# Autodesk Inventor assembly: Maintenance_stand
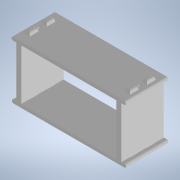
[picture p0: Inventor's stored thumbnail of the model, 180x180]
Saved by Autodesk Inventor 2020.2 (Build 242310000, 310)
## iProperties
Created: 2020-10-03
Part Number: Maintenance_stand
Document SubType Name: Assembly
Designer: touhu_zn72wdq
Author: touhu_zn72wdq
## Documents named in this file (3)
- C:\Users\touhu_zn72wdq\Documents\Inventor\Gankenkun_mente\Maintenance_stand.iam
- C:\Users\touhu_zn72wdq\Documents\Inventor\Gankenkun_mente\menteA.ipt
- C:\Users\touhu_zn72wdq\Documents\Inventor\Gankenkun_mente\menteB.ipt
## Components (4 placed, 2 different names)
1. menteA:1 — メイト:1, メイト:2, メイト:3, メイト:7, メイト:8, メイト:9
2. menteB:1 — メイト:1, メイト:2, メイト:3
3. menteA:2 — メイト:4, メイト:5, メイト:6
4. menteB:2 — メイト:4, メイト:5, メイト:6, メイト:7, メイト:8, メイト:9
## Relationships (9: Mate 9)
- メイト:1 [Mate]: menteA:1 ↔ menteB:1
- メイト:2 [Mate]: menteA:1 ↔ menteB:1
- メイト:3 [Mate]: menteA:1 ↔ menteB:1
- メイト:4 [Mate]: menteA:2 ↔ menteB:2
- メイト:5 [Mate]: menteA:2 ↔ menteB:2
- メイト:6 [Mate]: menteA:2 ↔ menteB:2
- メイト:7 [Mate]: menteA:1 ↔ menteB:2
- メイト:8 [Mate]: menteA:1 ↔ menteB:2
- メイト:9 [Mate]: menteA:1 ↔ menteB:2
